# Autodesk Inventor assembly: Back-Forth-Linkage
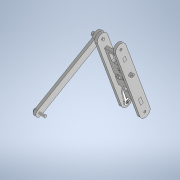
[picture p0: Inventor's stored thumbnail of the model, 180x180]
Saved by Autodesk Inventor 2022 (Build 260153000, 153)
## iProperties
Created: 2020-02-05
Part Number: Back-Forth-Linkage
Document SubType Name: Assembly
Designer: joshn
Author: joshn
Revision Number: NONE
## Documents named in this file (14)
- D:\Joshwin Emmanuel\Fab_accad\git_hub\Fab_Work\arm\step\part\Back-Forth-Linkage.iam
- D:\Joshwin Emmanuel\Fab_accad\git_hub\Fab_Work\arm\step\part\Main Arm Cross Web.ipt
- D:\Joshwin Emmanuel\Fab_accad\git_hub\Fab_Work\arm\step\part\Right Arm Base Joint.ipt
- D:\Joshwin Emmanuel\Fab_accad\git_hub\Fab_Work\arm\step\part\Left Arm Base Joint.ipt
- D:\Joshwin Emmanuel\Fab_accad\git_hub\Fab_Work\arm\step\part\Schraube _ Zylinder - M3,0 x 10,0_1.ipt
- D:\Joshwin Emmanuel\Fab_accad\git_hub\Fab_Work\arm\step\part\Right Wrist Joint.ipt
- D:\Joshwin Emmanuel\Fab_accad\git_hub\Fab_Work\arm\step\part\Mutter _  - M3,0 x 57,785_5.ipt
- D:\Joshwin Emmanuel\Fab_accad\git_hub\Fab_Work\arm\step\part\Mutter _  - M3,0 x 57,785_6.ipt
- D:\Joshwin Emmanuel\Fab_accad\git_hub\Fab_Work\arm\step\part\Zyl-Imbus M3x12_4.ipt
- D:\Joshwin Emmanuel\Fab_accad\git_hub\Fab_Work\arm\step\part\Zyl-Imbus M3x12_5.ipt
- D:\Joshwin Emmanuel\Fab_accad\git_hub\Fab_Work\arm\step\part\Schraube _ Kegelstumpf - M2,0 x 6,0_3.ipt
- D:\Joshwin Emmanuel\Fab_accad\git_hub\Fab_Work\arm\step\part\Schraube _ Kegelstumpf - M2,0 x 6,0_4.ipt
- D:\Joshwin Emmanuel\Fab_accad\git_hub\Fab_Work\arm\step\part\Schraube _ Zylinder - M3,0 x 10,0_2.ipt
- D:\Joshwin Emmanuel\Fab_accad\git_hub\Fab_Work\arm\step\part\SG90 - Micro Servo 9g - Tower Pro.2.ipt
## Components (13 placed, 9 different names)
1. Main Arm Cross Web
2. Right Arm Base Joint — Mate:2, Tangent:1, Mate:4
3. Left Arm Base Joint
4. Schraube : Zylinder - M3,0 x 10,0
5. Right Wrist Joint
6. Mutter :  - M3,0 x 57,785
7. Mutter :  - M3,0 x 57,785:1
8. Zyl-Imbus M3x12
9. Zyl-Imbus M3x12:1
10. Schraube : Kegelstumpf - M2,0 x 6,0 — Mate:3, Mate:4
11. Schraube : Kegelstumpf - M2,0 x 6,0:1 — Mate:1, Mate:5, Mate:6
12. Servo-Arm-zweiseitig — Mate:1, Mate:2, Tangent:1, Mate:3, Mate:5, Mate:6
13. Schraube : Zylinder - M3,0 x 10,0:1
## Relationships (7: Mate 6, Tangent 1)
- Mate:1: Schraube : Kegelstumpf - M2,0 x 6,0:1 ↔ Servo-Arm-zweiseitig
- Mate:2: Right Arm Base Joint ↔ Servo-Arm-zweiseitig
- Tangent:1: Right Arm Base Joint ↔ Servo-Arm-zweiseitig
- Mate:3: Schraube : Kegelstumpf - M2,0 x 6,0 ↔ Servo-Arm-zweiseitig
- Mate:4: Right Arm Base Joint ↔ Schraube : Kegelstumpf - M2,0 x 6,0
- Mate:5: Schraube : Kegelstumpf - M2,0 x 6,0:1 ↔ Servo-Arm-zweiseitig
- Mate:6: Schraube : Kegelstumpf - M2,0 x 6,0:1 ↔ Servo-Arm-zweiseitig
